# Autodesk Inventor assembly: Assembly1
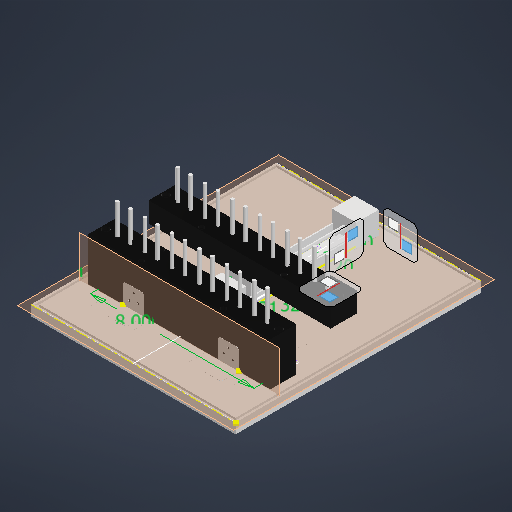
[picture p0: Inventor's stored thumbnail of the model, 512x512]
Saved by Autodesk Inventor 2026 (Build 300175000, 175)
## iProperties
Created: 2026-04-17
Part Number: Assembly1
Document SubType Name: Assembly
Designer: v.valentina
Author: v.valentina
## Documents named in this file (13)
- \\nfs.seas.wustl.edu\seaslab\home-lab\v.valentina\Documents\CADding Capstone\Assembly1.iam
- \\nfs.seas.wustl.edu\seaslab\home-lab\v.valentina\Documents\CADding Capstone\bases designs\OS_platform_0.5in.ipt
- \\nfs.seas.wustl.edu\seaslab\home-lab\v.valentina\Documents\Part1.ipt
- \\nfs.seas.wustl.edu\seaslab\home-lab\v.valentina\Documents\CADding Capstone\annas bases\Actuator Base.ipt
- \\nfs.seas.wustl.edu\seaslab\home-lab\v.valentina\Documents\CADding Capstone\annas bases\Lid.ipt
- \\nfs.seas.wustl.edu\seaslab\home-lab\v.valentina\Documents\CADding Capstone\annas bases\Stationary Base.ipt
- \\nfs.seas.wustl.edu\seaslab\home-lab\v.valentina\Documents\CADding Capstone\annas bases\dowel pins.ipt
- \\nfs.seas.wustl.edu\seaslab\home-lab\v.valentina\Documents\CADding Capstone\annas bases\lbrackets.ipt
- \\nfs.seas.wustl.edu\seaslab\home-lab\v.valentina\Documents\CADding Capstone\annas bases\l_bracket_large.ipt
- \\nfs.seas.wustl.edu\seaslab\home-lab\v.valentina\Documents\CADding Capstone\annas bases\Stationary Base_MIR.ipt
- \\nfs.seas.wustl.edu\seaslab\home-lab\v.valentina\Documents\CADding Capstone\annas bases\l_bracket_large_MIR.ipt
- \\nfs.seas.wustl.edu\seaslab\home-lab\v.valentina\Documents\CADding Capstone\annas bases\lbracket_short.ipt
- \\nfs.seas.wustl.edu\seaslab\home-lab\v.valentina\Documents\CADding Capstone\annas bases\lbracket_short_MIR.ipt
## Components (36 placed, 12 different names)
1. OS_platform_0.5in:1 — Mate:2, Mate:3, Mate:4, Flush:3, Flush:4, Mate:46, Mate:48, Mate:51, Mate:52, Mate:53
2. Part1:1 — Mate:51, Mate:52, Mate:53, Rigid:7
3. Stationary Base:1 — Mate:2, Rigid:2, Mate:3, Mate:4, Flush:3, Mate:5, Rigid:3, Mate:6, Mate:7, Rigid:4, Mate:9, Mate:10, Flush:5, Mate:47, Mate:49, Mate:54, Mate:55, Mate:56, Rigid:5, Rigid:6, Rigid:21
4. Lid:2 — Rigid:2
5. dowel pins:1 — Mate:5
6. dowel pins:2 — Rigid:3
7. dowel pins:3 — Mate:6, Rigid:5
8. dowel pins:4 — Mate:7
9. dowel pins:6 — Rigid:4
10. dowel pins:7 — Mate:9
11. dowel pins:8 — Mate:10
12. dowel pins:23 — Rigid:11
13. dowel pins:25 — Rigid:14
14. dowel pins:26 — Rigid:9
15. dowel pins:28 — Rigid:13
16. dowel pins:29 — Rigid:10
17. dowel pins:30 — Rigid:16
18. dowel pins:32 — Rigid:18
19. dowel pins:33 — Rigid:15
20. dowel pins:34 — Rigid:8
21. lbrackets:1 — Flush:4, Flush:5
22. l_bracket_large:2 — Mate:46, Mate:47
23. Stationary Base_MIR:1
24. l_bracket_large_MIR:1
25. lbracket_short:1 — Mate:48, Mate:49
26. lbracket_short_MIR:1
27. dowel pins:35 — Rigid:12
28. dowel pins:36 — Mate:55
29. dowel pins:38 — Rigid:6
30. dowel pins:40 — Rigid:17
31. dowel pins:41 — Mate:56
32. dowel pins:42 — Mate:54
33. Actuator Base:1 — Rigid:7, Rigid:8, Rigid:9, Rigid:10, Rigid:11, Rigid:12, Rigid:13, Rigid:14, Rigid:15, Rigid:16, Rigid:17, Rigid:18, Rigid:19, Rigid:20
34. Lid:3 — Rigid:20
35. dowel pins:43 — Rigid:19
36. dowel pins:44 — Rigid:21
## Relationships (41: WeldJoint 20, Mate 18, Flush 3)
- Mate:2: OS_platform_0.5in:1 ↔ Stationary Base:1
- Rigid:2 [WeldJoint]: Stationary Base:1 ↔ Lid:2
- Mate:3: OS_platform_0.5in:1 ↔ Stationary Base:1
- Mate:4: OS_platform_0.5in:1 ↔ Stationary Base:1
- Flush:3 (14 mm): OS_platform_0.5in:1 ↔ Stationary Base:1
- Mate:5: Stationary Base:1 ↔ dowel pins:1
- Rigid:3 [WeldJoint]: Stationary Base:1 ↔ dowel pins:2
- Mate:6: Stationary Base:1 ↔ dowel pins:3
- Mate:7: Stationary Base:1 ↔ dowel pins:4
- Rigid:4 [WeldJoint]: Stationary Base:1 ↔ dowel pins:6
- Mate:9: Stationary Base:1 ↔ dowel pins:7
- Mate:10: Stationary Base:1 ↔ dowel pins:8
- Flush:4: OS_platform_0.5in:1 ↔ lbrackets:1
- Flush:5: Stationary Base:1 ↔ lbrackets:1
- Mate:46: OS_platform_0.5in:1 ↔ l_bracket_large:2
- Mate:47: Stationary Base:1 ↔ l_bracket_large:2
- Mate:48: OS_platform_0.5in:1 ↔ lbracket_short:1
- Mate:49: Stationary Base:1 ↔ lbracket_short:1
- Mate:51: OS_platform_0.5in:1 ↔ Part1:1
- Mate:52 (112 mm): OS_platform_0.5in:1 ↔ Part1:1
- Mate:53 (15 mm): OS_platform_0.5in:1 ↔ Part1:1
- Mate:54: Stationary Base:1 ↔ dowel pins:42
- Mate:55: Stationary Base:1 ↔ dowel pins:36
- Mate:56: Stationary Base:1 ↔ dowel pins:41
- Rigid:5 [WeldJoint]: Stationary Base:1 ↔ dowel pins:3
- Rigid:6 [WeldJoint]: Stationary Base:1 ↔ dowel pins:38
- Rigid:7 [WeldJoint]: Part1:1 ↔ Actuator Base:1
- Rigid:8 [WeldJoint]: dowel pins:34 ↔ Actuator Base:1
- Rigid:9 [WeldJoint]: dowel pins:26 ↔ Actuator Base:1
- Rigid:10 [WeldJoint]: dowel pins:29 ↔ Actuator Base:1
- Rigid:11 [WeldJoint]: dowel pins:23 ↔ Actuator Base:1
- Rigid:12 [WeldJoint]: dowel pins:35 ↔ Actuator Base:1
- Rigid:13 [WeldJoint]: dowel pins:28 ↔ Actuator Base:1
- Rigid:14 [WeldJoint]: dowel pins:25 ↔ Actuator Base:1
- Rigid:15 [WeldJoint]: dowel pins:33 ↔ Actuator Base:1
- Rigid:16 [WeldJoint]: dowel pins:30 ↔ Actuator Base:1
- Rigid:17 [WeldJoint]: dowel pins:40 ↔ Actuator Base:1
- Rigid:18 [WeldJoint]: dowel pins:32 ↔ Actuator Base:1
- Rigid:19 [WeldJoint]: Actuator Base:1 ↔ dowel pins:43
- Rigid:20 [WeldJoint]: Actuator Base:1 ↔ Lid:3
- Rigid:21 [WeldJoint]: Stationary Base:1 ↔ dowel pins:44
